# Autodesk Inventor assembly: First FPV Drone
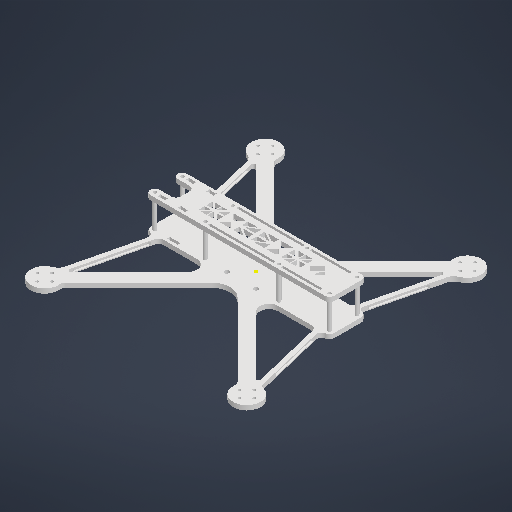
[picture p0: Inventor's stored thumbnail of the model, 512x512]
Saved by Autodesk Inventor 2026 (Build 300175050, 175E)
## iProperties
Created: 2025-07-14
Part Number: First FPV Drone
Document SubType Name: Assembly
Designer: User
Author: User
## Documents named in this file (4)
- E:\CAD\Parts\Drone\First FPV Drone.iam
- E:\CAD\Parts\Drone\Drone Frame 1.0.ipt
- E:\CAD\Parts\Drone\Beams.ipt
- E:\CAD\Parts\Drone\Top Of Drone.ipt
## Components (10 placed, 3 different names)
1. Drone Frame 1.0:1 — Rotational:1, Rotational:2, Rotational:3, Rotational:4, Rotational:5, Rotational:6, Rotational:7, Rotational:8
2. Beams:2 — Rotational:1
3. Beams:3 — Rotational:3, Mate:1
4. Beams:4 — Rotational:4
5. Beams:5 — Rotational:8, Mate:2
6. Beams:6 — Rotational:2
7. Beams:7 — Rotational:7
8. Beams:8 — Rotational:6
9. Beams:9 — Rotational:5
10. Top Of Drone:1 — Mate:1, Mate:2
## Relationships (10: RevoluteJoint 8, Mate 2)
- Rotational:1 [RevoluteJoint]: Drone Frame 1.0:1 ↔ Beams:2
- Rotational:2 [RevoluteJoint]: Drone Frame 1.0:1 ↔ Beams:6
- Rotational:3 [RevoluteJoint]: Drone Frame 1.0:1 ↔ Beams:3
- Rotational:4 [RevoluteJoint]: Drone Frame 1.0:1 ↔ Beams:4
- Rotational:5 [RevoluteJoint]: Drone Frame 1.0:1 ↔ Beams:9
- Rotational:6 [RevoluteJoint]: Drone Frame 1.0:1 ↔ Beams:8
- Rotational:7 [RevoluteJoint]: Drone Frame 1.0:1 ↔ Beams:7
- Rotational:8 [RevoluteJoint]: Drone Frame 1.0:1 ↔ Beams:5
- Mate:1: Beams:3 ↔ Top Of Drone:1
- Mate:2: Beams:5 ↔ Top Of Drone:1
